# Autodesk Inventor assembly: P1704_E1
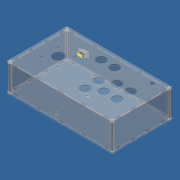
[picture p0: Inventor's stored thumbnail of the model, 180x180]
Saved by Autodesk Inventor 2015 (Build 190159000, 159)
## iProperties
Created: 2018-05-07
Part Number: P1704_E1
Project: Manette arcade
Description: Manette
Document SubType Name: Assembly
Designer: Alexandre.PICOTTE
Author: Alexandre.PICOTTE
## Documents named in this file (9)
- C:\Users\Alexandre.PICOTTE\Documents\P1704_Manettes\06_Dessins\Manette_arcade\P1704_E1_Manette.iam
- C:\Users\Alexandre.PICOTTE\Documents\P1704_Manettes\06_Dessins\Manette_arcade\P1704_006_Socle.ipt
- C:\Users\Alexandre.PICOTTE\Documents\P1704_Manettes\06_Dessins\Manette_arcade\P1704_005_Paroi_latérale.ipt
- C:\Users\Alexandre.PICOTTE\Documents\P1704_Manettes\06_Dessins\Manette_arcade\P1704_003_Paroi_avant.ipt
- C:\Users\Alexandre.PICOTTE\Documents\P1704_Manettes\06_Dessins\Manette_arcade\P1704_004_Paroi_arrière.ipt
- C:\Users\Alexandre.PICOTTE\Documents\P1704_Manettes\06_Dessins\Manette_arcade\P1704_002_Toiture.ipt
- C:\Users\Alexandre.PICOTTE\Documents\Inventor\Content Center Files\R2015\fr-FR\D-Sub Male Crimp\D-Sub Male Crimp 9CKT.ipt
- C:\Users\Alexandre.PICOTTE\Documents\P1704_Manettes\06_Dessins\Manette_arcade\P1704_001_Pied.ipt
- C:\Users\Alexandre.PICOTTE\Documents\Inventor\Content Center Files\R2015\fr-FR\ISO 4762(2)\ISO 4762 - M3 x 5ISO.ipt
## Components (21 placed, 8 different names)
1. P1704_006_Socle:1 — Affleurement:1, Placage:1, Placage:2, Affleurement:2, Placage:3, Placage:4, Placage:5, Placage:6, Placage:7, Placage:8, Placage:9, Placage:10, Logement:9, Logement:10, Logement:11, Logement:12, Logement:13, Logement:14
2. P1704_005_Paroi_latérale:1 — Affleurement:1, Placage:1, Placage:2, Placage:12, Placage:13
3. P1704_005_Paroi_latérale:2 — Affleurement:2, Placage:3, Placage:4
4. P1704_003_Paroi_avant:1 — Placage:5, Placage:6, Placage:7, Placage:11
5. P1704_004_Paroi_arrière:1 — Placage:8, Placage:9, Placage:10, Placage:14, Placage:15
6. P1704_002_Toiture:1 — Placage:11, Placage:12, Placage:13, Logement:1, Logement:2, Logement:3, Logement:4, Logement:5, Logement:6, Logement:7, Logement:8, Angle:1
7. P1704_001_Pied:1 — Logement:2
8. P1704_001_Pied:2 — Logement:4
9. P1704_001_Pied:3 — Logement:1
10. P1704_001_Pied:4 — Logement:3
11. ISO 4762 M3 x 5:1 — Logement:5
12. ISO 4762 M3 x 5:2 — Logement:6
13. ISO 4762 M3 x 5:3 — Logement:7
14. ISO 4762 M3 x 5:4 — Logement:8
15. ISO 4762 M3 x 5:5 — Logement:9
16. ISO 4762 M3 x 5:6 — Logement:10
17. ISO 4762 M3 x 5:7 — Logement:11
18. ISO 4762 M3 x 5:8 — Logement:12
19. ISO 4762 M3 x 5:9 — Logement:13
20. ISO 4762 M3 x 5:10 — Logement:14
21. Sertissage mâle D-Sub D-Sub Male Crimp 9CKT:1 — Placage:14, Angle:1, Placage:15
## Relationships (32: Mate 15, Insert 14, Flush 2, Angle 1)
- Affleurement:1 [Flush]: P1704_006_Socle:1 ↔ P1704_005_Paroi_latérale:1
- Placage:1 [Mate]: P1704_006_Socle:1 ↔ P1704_005_Paroi_latérale:1
- Placage:2 [Mate]: P1704_006_Socle:1 ↔ P1704_005_Paroi_latérale:1
- Affleurement:2 [Flush]: P1704_006_Socle:1 ↔ P1704_005_Paroi_latérale:2
- Placage:3 [Mate]: P1704_006_Socle:1 ↔ P1704_005_Paroi_latérale:2
- Placage:4 [Mate]: P1704_006_Socle:1 ↔ P1704_005_Paroi_latérale:2
- Placage:5 [Mate]: P1704_006_Socle:1 ↔ P1704_003_Paroi_avant:1
- Placage:6 [Mate]: P1704_006_Socle:1 ↔ P1704_003_Paroi_avant:1
- Placage:7 [Mate]: P1704_006_Socle:1 ↔ P1704_003_Paroi_avant:1
- Placage:8 [Mate]: P1704_006_Socle:1 ↔ P1704_004_Paroi_arrière:1
- Placage:9 [Mate]: P1704_006_Socle:1 ↔ P1704_004_Paroi_arrière:1
- Placage:10 [Mate]: P1704_006_Socle:1 ↔ P1704_004_Paroi_arrière:1
- Placage:11 [Mate]: P1704_003_Paroi_avant:1 ↔ P1704_002_Toiture:1
- Placage:12 [Mate]: P1704_005_Paroi_latérale:1 ↔ P1704_002_Toiture:1
- Placage:13 [Mate]: P1704_005_Paroi_latérale:1 ↔ P1704_002_Toiture:1
- Logement:1 [Insert]: P1704_002_Toiture:1 ↔ P1704_001_Pied:3
- Logement:2 [Insert]: P1704_002_Toiture:1 ↔ P1704_001_Pied:1
- Logement:3 [Insert]: P1704_002_Toiture:1 ↔ P1704_001_Pied:4
- Logement:4 [Insert]: P1704_002_Toiture:1 ↔ P1704_001_Pied:2
- Logement:5 [Insert]: P1704_002_Toiture:1 ↔ ISO 4762 M3 x 5:1
- Logement:6 [Insert]: P1704_002_Toiture:1 ↔ ISO 4762 M3 x 5:2
- Logement:7 [Insert]: P1704_002_Toiture:1 ↔ ISO 4762 M3 x 5:3
- Logement:8 [Insert]: P1704_002_Toiture:1 ↔ ISO 4762 M3 x 5:4
- Logement:9 [Insert]: P1704_006_Socle:1 ↔ ISO 4762 M3 x 5:5
- Logement:10 [Insert]: P1704_006_Socle:1 ↔ ISO 4762 M3 x 5:6
- Logement:11 [Insert]: P1704_006_Socle:1 ↔ ISO 4762 M3 x 5:7
- Logement:12 [Insert]: P1704_006_Socle:1 ↔ ISO 4762 M3 x 5:8
- Logement:13 [Insert]: P1704_006_Socle:1 ↔ ISO 4762 M3 x 5:9
- Logement:14 [Insert]: P1704_006_Socle:1 ↔ ISO 4762 M3 x 5:10
- Placage:14 [Mate]: P1704_004_Paroi_arrière:1 ↔ Sertissage mâle D-Sub D-Sub Male Crimp 9CKT:1
- Angle:1 (0 deg): P1704_002_Toiture:1 ↔ Sertissage mâle D-Sub D-Sub Male Crimp 9CKT:1
- Placage:15 [Mate]: P1704_004_Paroi_arrière:1 ↔ Sertissage mâle D-Sub D-Sub Male Crimp 9CKT:1
